# Autodesk Inventor assembly: Lift.00.00.00.00
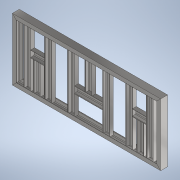
[picture p0: Inventor's stored thumbnail of the model, 180x180]
Saved by Autodesk Inventor 2021 (Build 250183000, 183)
## iProperties
Created: 2020-09-20
Part Number: Lift.00.00.00.00
Document SubType Name: Assembly
Designer: Kostya
_SolveAssemblyDoc: Frame Generator Solve Assembly
_Version: 25.0.0
Author: Kostya
## Documents named in this file (3)
- C:\Lift\Lift.00.00.00.00.iam
- C:\Lift\Lift.00.00.00.08.ipt
- C:\Lift\Lift.00.00.00.00\Frame\Frame 1600626060237.iam
## Components (2 placed, 2 different names)
1. Lift.00.00.00.08:1 — Совмещение:1, Совмещение:2, Заподлицо:1
2. Frame 1600626060237:1 [sub-assembly]
## Relationships (3: Mate 2, Flush 1)
- Совмещение:1 [Mate]: Lift.00.00.00.08:1
- Совмещение:2 [Mate]: Lift.00.00.00.08:1
- Заподлицо:1 [Flush]: Lift.00.00.00.08:1
